# Autodesk Inventor assembly: ENSAMBLE CALDERIN ACH-62L-2021-P JP2021-108
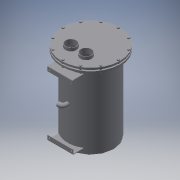
[picture p0: Inventor's stored thumbnail of the model, 180x180]
Saved by Autodesk Inventor 2017 (Build 210142000, 142)
## iProperties
Created: 2021-06-11
Part Number: ENSAMBLE CALDERIN ACH-62L-2021-P JP2021-108
Document SubType Name: Assembly
Designer: USUARIO
Author: USUARIO
Revision Number: ANY
## Documents named in this file (12)
- D:\Laboratorio\Autoclave\Autoclave Horizontal\Con Precamara\2021\Autoclave 62L Dempharma SAS OP2021108 #0045885XX\Modelo\ENSAMBLE CALDERIN ACH-62L-2021-P JP2021-108.iam
- D:\Laboratorio\Autoclave\Autoclave Horizontal\Con Precamara\2021\Autoclave 62L Dempharma SAS OP2021108 #0045885XX\Modelo\CUERPO CALDERIN ACH-62L-2021-P JP2021-108_Predeterminado_Como mecanizada_.ipt
- D:\Laboratorio\Autoclave\Autoclave Horizontal\Con Precamara\2021\Autoclave 62L Dempharma SAS OP2021108 #0045885XX\Modelo\FONDO CALDERIN ACH-62L-2021-P JP2021-108.ipt
- D:\Laboratorio\Autoclave\Autoclave Horizontal\Con Precamara\2021\Autoclave 62L Dempharma SAS OP2021108 #0045885XX\Modelo\FLANCHE CALDERIN ACH-62L-2021-P JP2021-108.ipt
- D:\Laboratorio\Autoclave\Autoclave Horizontal\Con Precamara\2021\Autoclave 62L Dempharma SAS OP2021108 #0045885XX\Modelo\TAPA CALDERIN ACH-62L-2021-P JP2021-108.ipt
- D:\Laboratorio\Autoclave\Autoclave Horizontal\Con Precamara\2021\Autoclave 62L Dempharma SAS OP2021108 #0045885XX\Modelo\SOPORTE CALDERIN ACH-62L-2021-P JP2021-108.ipt
- D:\Laboratorio\Autoclave\Autoclave Horizontal\Con Precamara\2021\Autoclave 62L Dempharma SAS OP2021108 #0045885XX\Modelo\UNION LISA 1-2.ipt
- D:\Laboratorio\Autoclave\Autoclave Horizontal\Con Precamara\2021\Autoclave 62L Dempharma SAS OP2021108 #0045885XX\Modelo\UNION LISA 1-4.ipt
- D:\Laboratorio\Autoclave\Autoclave Horizontal\Con Precamara\2021\Autoclave 62L Dempharma SAS OP2021108 #0045885XX\Modelo\UNION LISA 2.ipt
- D:\Laboratorio\Autoclave\Autoclave Horizontal\Con Precamara\2021\Autoclave 62L Dempharma SAS OP2021108 #0045885XX\Modelo\CODO 1-2.ipt
- D:\Laboratorio\Autoclave\Autoclave Horizontal\Con Precamara\2021\Autoclave 62L Dempharma SAS OP2021108 #0045885XX\Modelo\EMPAQUE CALDERIN ACH-62L-2021-P JP2021-108.ipt
- D:\Laboratorio\Autoclave\Autoclave Horizontal\Con Precamara\2021\Autoclave 62L Dempharma SAS OP2021108 #0045885XX\Modelo\hex bolt_ai_PreviewCfg.ipt
## Components (30 placed, 30 different names)
1. CUERPO CALDERIN ACH-62L-2021-P JP2021-108_Predeterminado<Como mecanizada>_64 — Mate:1
2. FONDO CALDERIN ACH-62L-2021-P JP2021-108_65
3. FLANCHE CALDERIN ACH-62L-2021-P JP2021-108_66
4. TAPA CALDERIN ACH-62L-2021-P JP2021-108_67
5. SOPORTE CALDERIN ACH-62L-2021-P JP2021-108_68
6. SOPORTE CALDERIN ACH-62L-2021-P JP2021-108_69
7. UNION LISA 1-2_70
8. UNION LISA 1-4_71
9. UNION LISA 2_72
10. CODO 1-2_73 — Mate:1
11. UNION LISA 2_74
12. UNION LISA 1-4_75
13. UNION LISA 1-4_76
14. UNION LISA 1-2_77
15. UNION LISA 1-2_78
16. EMPAQUE CALDERIN ACH-62L-2021-P JP2021-108_79
17. hex bolt_ai_PreviewCfg_80
18. hex bolt_ai_PreviewCfg_81
19. hex bolt_ai_PreviewCfg_82
20. hex bolt_ai_PreviewCfg_83
21. hex bolt_ai_PreviewCfg_84
22. hex bolt_ai_PreviewCfg_85
23. hex bolt_ai_PreviewCfg_86
24. hex bolt_ai_PreviewCfg_87
25. hex bolt_ai_PreviewCfg_88
26. hex bolt_ai_PreviewCfg_89
27. hex bolt_ai_PreviewCfg_90
28. hex bolt_ai_PreviewCfg_91
29. UNION LISA 1-4_92
30. UNION LISA 1-4_93
## Relationships (1: Mate 1)
- Mate:1: CUERPO CALDERIN ACH-62L-2021-P JP2021-108_Predeterminado<Como mecanizada>_64 ↔ CODO 1-2_73
